# Autodesk Inventor assembly: Body_as
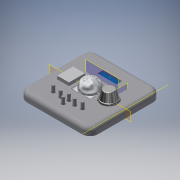
[picture p0: Inventor's stored thumbnail of the model, 180x180]
Saved by Autodesk Inventor 2017 (Build 210142000, 142)
## iProperties
Created: 2017-02-21
Part Number: Body_as
Document SubType Name: Assembly
Designer: prosp
Author: prosp
## Documents named in this file (7)
- D:\GitHub\Smart_Unit\Body_as.iam
- D:\GitHub\Smart_Unit\Body.ipt
- D:\GitHub\Smart_Unit\MotionSensor.ipt
- D:\GitHub\Smart_Unit\CO2_Sensor.ipt
- D:\GitHub\Smart_Unit\DHT22.ipt
- D:\GitHub\Smart_Unit\OLED_128x32.ipt
- D:\GitHub\Smart_Unit\Keyboard1.ipt
## Components (6 placed, 6 different names)
1. Body:1 — Mate:2, Mate:5, Mate:8, Mate:9, Mate:10, Mate:11, Mate:12, Flush:1, Flush:2, Mate:14, Mate:15, Mate:17, Mate:18, Flush:3
2. MotionSensor:1 — Mate:1, Mate:8, Mate:9, Flush:1, Flush:2, Mate:16
3. CO2_Sensor:1 — Mate:14, Mate:16, Mate:17
4. DHT22:1 — Mate:10, Mate:11, Mate:12, Mate:19
5. OLED_128x32:1 — Angle:1, Mate:2, Mate:5, Mate:15
6. Keyboard1:1 — Mate:18, Flush:3, Mate:19
## Relationships (18: Mate 14, Flush 3, Angle 1)
- Mate:1: MotionSensor:1
- Angle:1 (0 deg): OLED_128x32:1
- Mate:2 (11 mm): Body:1 ↔ OLED_128x32:1
- Mate:5 (24.5 mm): Body:1 ↔ OLED_128x32:1
- Mate:8 (27 mm): Body:1 ↔ MotionSensor:1
- Mate:9 (31.25 mm): Body:1 ↔ MotionSensor:1
- Mate:10 (33 mm): Body:1 ↔ DHT22:1
- Mate:11 (59.5 mm): Body:1 ↔ DHT22:1
- Mate:12 (1 mm): Body:1 ↔ DHT22:1
- Flush:1: Body:1 ↔ MotionSensor:1
- Flush:2: Body:1 ↔ MotionSensor:1
- Mate:14 (1 mm): Body:1 ↔ CO2_Sensor:1
- Mate:15: Body:1 ↔ OLED_128x32:1
- Mate:16 (2.2606 mm): MotionSensor:1 ↔ CO2_Sensor:1
- Mate:17: Body:1 ↔ CO2_Sensor:1
- Mate:18: Body:1 ↔ Keyboard1:1
- Flush:3: Body:1 ↔ Keyboard1:1
- Mate:19 (0.5 mm): DHT22:1 ↔ Keyboard1:1
